# Autodesk Inventor assembly: trailer
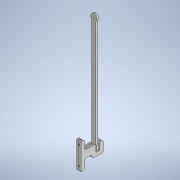
[picture p0: Inventor's stored thumbnail of the model, 180x180]
Saved by Autodesk Inventor 2020 (Build 240168000, 168)
## iProperties
Created: 2020-03-17
Part Number: trailer
Document SubType Name: Assembly
Designer: erwin
Author: erwin
## Documents named in this file (4)
- D:\GitHub\BeachMaid\platform-2\trailer\trailer.iam
- D:\GitHub\BeachMaid\platform-2\trailer\clamp.ipt
- D:\GitHub\BeachMaid\platform-2\trailer\clamp_MIR.ipt
- D:\GitHub\BeachMaid\platform-2\trailer\arm.ipt
## Components (3 placed, 3 different names)
1. clamp:1 — Flush:1, Flush:2
2. clamp_MIR:1
3. arm:1 — Flush:1, Flush:2
## Relationships (2: Flush 2)
- Flush:1: clamp:1 ↔ arm:1
- Flush:2: clamp:1 ↔ arm:1
